# Autodesk Inventor assembly: Caja CNAF
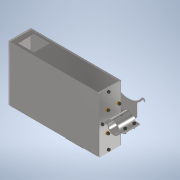
[picture p0: Inventor's stored thumbnail of the model, 180x180]
Saved by Autodesk Inventor 2020.3 (Build 243373000, 373)
## iProperties
Created: 2020-06-30
Part Number: Caja CNAF
Document SubType Name: Assembly
Designer: Bruno
Author: Bruno
## Documents named in this file (14)
- C:\Users\Bruno\Desktop\CNAF\CNAF-3\Caja CNAF.iam
- C:\Users\Bruno\Desktop\CNAF\CNAF-3\base_v7.ipt
- C:\Users\Bruno\Desktop\CNAF\CNAF-3\tapa_v7.ipt
- C:\Users\Bruno\Desktop\CNAF\CNAF-3\Tuerca Remachable M4.ipt
- C:\Users\Bruno\Desktop\CNAF\CNAF-3\Perno Parker DIN912 M4x0.7x10-8.8.ipt
- C:\Users\Bruno\Desktop\CNAF\CNAF-3\Perno Parker DIN912 M4x0.7x40-8.8.ipt
- C:\Users\Bruno\Desktop\CNAF\CNAF-3\Sello Plato Oring 2-343.ipt
- C:\Users\Bruno\Desktop\CNAF\CNAF-3\Plato Calefactor.ipt
- C:\Users\Bruno\Desktop\CNAF\CNAF-3\Barra fijación calefactor V2.ipt
- C:\Users\Bruno\Desktop\CNAF\CNAF-3\Tuerca DIN934-M4.ipt
- C:\Users\Bruno\Desktop\CNAF\CNAF-3\Sujetador Vaso.ipt
- C:\Users\Bruno\Desktop\CNAF\CNAF-3\Sujetador Porta Suero.iam
- C:\Users\Bruno\Desktop\CNAF\CNAF-3\Arandela Presion DIN127B D4.ipt
- C:\Users\Bruno\Desktop\CNAF\CNAF-3\Prisionero DIN913-M5x5.ipt
## Components (52 placed, 13 different names)
1. base_v7:1 — Mate:1, Flush:1, Flush:2, Cylindrical:1, Cylindrical:2, Cylindrical:3, Cylindrical:4, Cylindrical:5, Cylindrical:6, Cylindrical:7, Cylindrical:8, Cylindrical:9, Cylindrical:10, Cylindrical:28, Cylindrical:29
2. tapa_v7:1 — Mate:1, Flush:1, Flush:2, Cylindrical:11, Cylindrical:12, Cylindrical:13, Cylindrical:14, Cylindrical:15, Cylindrical:16, Cylindrical:17, Cylindrical:18, Cylindrical:19, Cylindrical:20, Rotational:1, Rotational:2, Cylindrical:21, Cylindrical:33, Cylindrical:34, Cylindrical:35, Cylindrical:36
3. Tuerca Remachable M4:1 — Cylindrical:1
4. Tuerca Remachable M4:2 — Cylindrical:4
5. Tuerca Remachable M4:3 — Cylindrical:2
6. Tuerca Remachable M4:4 — Cylindrical:3
7. Tuerca Remachable M4:5 — Cylindrical:7
8. Tuerca Remachable M4:6 — Cylindrical:6
9. Tuerca Remachable M4:7 — Cylindrical:5
10. Tuerca Remachable M4:8 — Cylindrical:10
11. Tuerca Remachable M4:9 — Cylindrical:9
12. Tuerca Remachable M4:10 — Cylindrical:8
13. Perno Parker DIN912 M4x0.7x10-8.8:1 — Cylindrical:11
14. Perno Parker DIN912 M4x0.7x10-8.8:2 — Cylindrical:13
15. Perno Parker DIN912 M4x0.7x10-8.8:3 — Cylindrical:12
16. Perno Parker DIN912 M4x0.7x10-8.8:4 — Cylindrical:14
17. Perno Parker DIN912 M4x0.7x10-8.8:5 — Cylindrical:15
18. Perno Parker DIN912 M4x0.7x10-8.8:6 — Cylindrical:16
19. Perno Parker DIN912 M4x0.7x10-8.8:7 — Cylindrical:17
20. Perno Parker DIN912 M4x0.7x10-8.8:8 — Cylindrical:20
21. Perno Parker DIN912 M4x0.7x10-8.8:9 — Cylindrical:19
22. Perno Parker DIN912 M4x0.7x10-8.8:10 — Cylindrical:18
23. Perno Parker DIN912 M4x0.7x40-8.8:1 — Rotational:1
24. Perno Parker DIN912 M4x0.7x40-8.8:2 — Rotational:2, Insert:1
25. Sello Plato Oring 2-343:1 — Cylindrical:21, Cylindrical:22
26. Plato Calefactor:1 — Cylindrical:22, Cylindrical:58, Cylindrical:59
27. Barra fijación calefactor V2:1 — Insert:1, Cylindrical:23, Cylindrical:24
28. Tuerca DIN934-M4:1 — Cylindrical:23
29. Tuerca DIN934-M4:2 — Cylindrical:24
30. Tuerca Remachable M4:11 — Cylindrical:28
31. Tuerca Remachable M4:12 — Cylindrical:29, Cylindrical:49
32. Perno Parker DIN912 M4x0.7x10-8.8:11 — Cylindrical:51
33. Perno Parker DIN912 M4x0.7x10-8.8:12 — Cylindrical:50
34. Tuerca Remachable M4:13 — Cylindrical:33
35. Tuerca Remachable M4:14 — Cylindrical:34, Cylindrical:37
36. Tuerca Remachable M4:15 — Cylindrical:35, Cylindrical:38
37. Tuerca Remachable M4:16 — Cylindrical:36
38. Sujetador Porta Suero:1 [sub-assembly] — Cylindrical:37, Cylindrical:39, Cylindrical:40, Cylindrical:52, Cylindrical:53
39. Sujetador Porta Suero:2 [sub-assembly] — Cylindrical:38, Cylindrical:41, Cylindrical:42, Cylindrical:54, Cylindrical:55
40. Perno Parker DIN912 M4x0.7x10-8.8:13 — Cylindrical:39
41. Perno Parker DIN912 M4x0.7x10-8.8:14 — Cylindrical:40
42. Perno Parker DIN912 M4x0.7x10-8.8:15 — Cylindrical:42
43. Perno Parker DIN912 M4x0.7x10-8.8:16 — Cylindrical:41
44. Sujetador Vaso:1 — Cylindrical:49, Cylindrical:50, Cylindrical:51
45. Arandela Presion DIN127B D4:1 — Cylindrical:52, Cylindrical:57
46. Arandela Presion DIN127B D4:2 — Cylindrical:53, Cylindrical:56
47. Tuerca DIN934-M4:3 — Cylindrical:54
48. Tuerca DIN934-M4:4 — Cylindrical:55
49. Perno Parker DIN912 M4x0.7x10-8.8:17 — Cylindrical:57
50. Perno Parker DIN912 M4x0.7x10-8.8:18 — Cylindrical:56
51. Prisionero DIN913-M5x5:1 — Cylindrical:59
52. Prisionero DIN913-M5x5:2 — Cylindrical:58
## Relationships (53: CylindricalJoint 47, Flush 2, RevoluteJoint 2, Mate 1, Insert 1)
- Mate:1 (1 mm): base_v7:1 ↔ tapa_v7:1
- Flush:1 (1 mm): base_v7:1 ↔ tapa_v7:1
- Flush:2: base_v7:1 ↔ tapa_v7:1
- Cylindrical:1: base_v7:1 ↔ Tuerca Remachable M4:1
- Cylindrical:2: base_v7:1 ↔ Tuerca Remachable M4:3
- Cylindrical:3: base_v7:1 ↔ Tuerca Remachable M4:4
- Cylindrical:4: base_v7:1 ↔ Tuerca Remachable M4:2
- Cylindrical:5: base_v7:1 ↔ Tuerca Remachable M4:7
- Cylindrical:6: base_v7:1 ↔ Tuerca Remachable M4:6
- Cylindrical:7: base_v7:1 ↔ Tuerca Remachable M4:5
- Cylindrical:8: base_v7:1 ↔ Tuerca Remachable M4:10
- Cylindrical:9: base_v7:1 ↔ Tuerca Remachable M4:9
- Cylindrical:10: base_v7:1 ↔ Tuerca Remachable M4:8
- Cylindrical:11: tapa_v7:1 ↔ Perno Parker DIN912 M4x0.7x10-8.8:1
- Cylindrical:12: tapa_v7:1 ↔ Perno Parker DIN912 M4x0.7x10-8.8:3
- Cylindrical:13: tapa_v7:1 ↔ Perno Parker DIN912 M4x0.7x10-8.8:2
- Cylindrical:14: tapa_v7:1 ↔ Perno Parker DIN912 M4x0.7x10-8.8:4
- Cylindrical:15: tapa_v7:1 ↔ Perno Parker DIN912 M4x0.7x10-8.8:5
- Cylindrical:16: tapa_v7:1 ↔ Perno Parker DIN912 M4x0.7x10-8.8:6
- Cylindrical:17: tapa_v7:1 ↔ Perno Parker DIN912 M4x0.7x10-8.8:7
- Cylindrical:18: tapa_v7:1 ↔ Perno Parker DIN912 M4x0.7x10-8.8:10
- Cylindrical:19: tapa_v7:1 ↔ Perno Parker DIN912 M4x0.7x10-8.8:9
- Cylindrical:20: tapa_v7:1 ↔ Perno Parker DIN912 M4x0.7x10-8.8:8
- Rotational:1 [RevoluteJoint]: tapa_v7:1 ↔ Perno Parker DIN912 M4x0.7x40-8.8:1
- Rotational:2 [RevoluteJoint]: tapa_v7:1 ↔ Perno Parker DIN912 M4x0.7x40-8.8:2
- Cylindrical:21: tapa_v7:1 ↔ Sello Plato Oring 2-343:1
- Cylindrical:22: Sello Plato Oring 2-343:1 ↔ Plato Calefactor:1
- Insert:1 (10.67 mm): Perno Parker DIN912 M4x0.7x40-8.8:2 ↔ Barra fijación calefactor V2:1
- Cylindrical:23: Barra fijación calefactor V2:1 ↔ Tuerca DIN934-M4:1
- Cylindrical:24: Barra fijación calefactor V2:1 ↔ Tuerca DIN934-M4:2
- Cylindrical:28: base_v7:1 ↔ Tuerca Remachable M4:11
- Cylindrical:29: base_v7:1 ↔ Tuerca Remachable M4:12
- Cylindrical:33: tapa_v7:1 ↔ Tuerca Remachable M4:13
- Cylindrical:34: tapa_v7:1 ↔ Tuerca Remachable M4:14
- Cylindrical:35: tapa_v7:1 ↔ Tuerca Remachable M4:15
- Cylindrical:36: tapa_v7:1 ↔ Tuerca Remachable M4:16
- Cylindrical:37: Tuerca Remachable M4:14 ↔ Sujetador Porta Suero:1
- Cylindrical:38: Tuerca Remachable M4:15 ↔ Sujetador Porta Suero:2
- Cylindrical:39: Sujetador Porta Suero:1 ↔ Perno Parker DIN912 M4x0.7x10-8.8:13
- Cylindrical:40: Sujetador Porta Suero:1 ↔ Perno Parker DIN912 M4x0.7x10-8.8:14
- Cylindrical:41: Sujetador Porta Suero:2 ↔ Perno Parker DIN912 M4x0.7x10-8.8:16
- Cylindrical:42: Sujetador Porta Suero:2 ↔ Perno Parker DIN912 M4x0.7x10-8.8:15
- Cylindrical:49: Tuerca Remachable M4:12 ↔ Sujetador Vaso:1
- Cylindrical:50: Perno Parker DIN912 M4x0.7x10-8.8:12 ↔ Sujetador Vaso:1
- Cylindrical:51: Perno Parker DIN912 M4x0.7x10-8.8:11 ↔ Sujetador Vaso:1
- Cylindrical:52: Sujetador Porta Suero:1 ↔ Arandela Presion DIN127B D4:1
- Cylindrical:53: Sujetador Porta Suero:1 ↔ Arandela Presion DIN127B D4:2
- Cylindrical:54: Sujetador Porta Suero:2 ↔ Tuerca DIN934-M4:3
- Cylindrical:55: Sujetador Porta Suero:2 ↔ Tuerca DIN934-M4:4
- Cylindrical:56: Arandela Presion DIN127B D4:2 ↔ Perno Parker DIN912 M4x0.7x10-8.8:18
- Cylindrical:57: Arandela Presion DIN127B D4:1 ↔ Perno Parker DIN912 M4x0.7x10-8.8:17
- Cylindrical:58: Plato Calefactor:1 ↔ Prisionero DIN913-M5x5:2
- Cylindrical:59: Plato Calefactor:1 ↔ Prisionero DIN913-M5x5:1
